# Autodesk Inventor assembly: Assembly
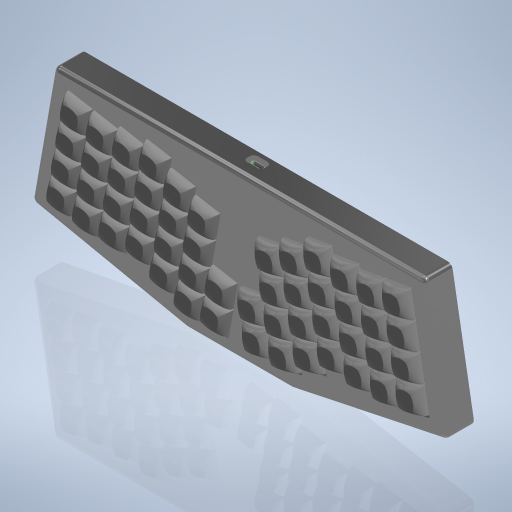
[picture p0: Inventor's stored thumbnail of the model, 512x512]
Saved by Autodesk Inventor 2023 (Build 270158000, 158)
## iProperties
Part Number: Assembly
Document SubType Name: Assembly
Designer: hainguyen
Author: hainguyen
## Documents named in this file (10)
- C:\Users\hainguyen\Documents\Inventor\atreus-52\Assembly.iam
- C:\Users\hainguyen\Documents\Inventor\atreus-52\atreus52_hotswap.ipt
- C:\Users\hainguyen\Documents\Inventor\atreus-52\Kailh Hotswap.ipt
- C:\Users\hainguyen\Documents\Inventor\atreus-52\asm_mx_asm_PLATE.ipt
- C:\Users\hainguyen\Documents\Inventor\atreus-52\DSA 1u.ipt
- C:\Users\hainguyen\Documents\Inventor\atreus-52\pattern.ipt
- C:\Users\hainguyen\Documents\Inventor\atreus-52\switch-plates.ipt
- C:\Users\hainguyen\Documents\Inventor\atreus-52\HRO_TYPE-C-31-M-12.ipt
- C:\Users\hainguyen\Documents\Inventor\atreus-52\bottom-case.ipt
- C:\Users\hainguyen\Documents\Inventor\atreus-52\top-case.ipt
## Components (162 placed, 9 different names)
1. atreus52_hotswap:1 — Mate:1, Mate:2, Mate:3, Mate:4, Mate:5, Angle:1, Mate:9, Mate:10, Mate:11, Mate:12, Mate:13, Angle:2, Flush:3, Mate:21, Mate:22
2. pattern:1 — Flush:1, Flush:2
3. switch-plates:1 — Mate:19, Mate:20, Flush:4
4. HRO_TYPE-C-31-M-12:1 — Flush:3, Mate:21, Mate:22
5. bottom-case:1 — Flush:4, Mate:23
6. top-case:1 — Mate:23
7. Kailh Hotswap:1 — Mate:1, Mate:2, Mate:3, Flush:1
8. asm_mx_asm_PLATE:1 — Mate:4, Mate:5, Angle:1, Mate:6, Mate:7, Mate:8
9. DSA 1u:1 — Mate:6, Mate:7, Mate:8
10. Kailh Hotswap:2
11. asm_mx_asm_PLATE:2
12. DSA 1u:2
13. Kailh Hotswap:3
14. asm_mx_asm_PLATE:3
15. DSA 1u:3
16. Kailh Hotswap:4
17. asm_mx_asm_PLATE:4
18. DSA 1u:4
19. Kailh Hotswap:5
20. asm_mx_asm_PLATE:5
21. DSA 1u:5
22. Kailh Hotswap:6
23. asm_mx_asm_PLATE:6
24. DSA 1u:6
25. Kailh Hotswap:7
26. asm_mx_asm_PLATE:7
27. DSA 1u:7
28. Kailh Hotswap:8
29. asm_mx_asm_PLATE:8
30. DSA 1u:8
31. Kailh Hotswap:9
32. asm_mx_asm_PLATE:9
33. DSA 1u:9
34. Kailh Hotswap:10
35. asm_mx_asm_PLATE:10
36. DSA 1u:10
37. Kailh Hotswap:11
38. asm_mx_asm_PLATE:11
39. DSA 1u:11
40. Kailh Hotswap:12
41. asm_mx_asm_PLATE:12
42. DSA 1u:12
43. Kailh Hotswap:13
44. asm_mx_asm_PLATE:13
45. DSA 1u:13
46. Kailh Hotswap:14
47. asm_mx_asm_PLATE:14
48. DSA 1u:14
49. Kailh Hotswap:15
50. asm_mx_asm_PLATE:15
51. DSA 1u:15
52. Kailh Hotswap:16
53. asm_mx_asm_PLATE:16
54. DSA 1u:16
55. Kailh Hotswap:17
56. asm_mx_asm_PLATE:17
57. DSA 1u:17
58. Kailh Hotswap:18
59. asm_mx_asm_PLATE:18
60. DSA 1u:18
61. Kailh Hotswap:19
62. asm_mx_asm_PLATE:19
63. DSA 1u:19
64. Kailh Hotswap:20
65. asm_mx_asm_PLATE:20
66. DSA 1u:20
67. Kailh Hotswap:21
68. asm_mx_asm_PLATE:21
69. DSA 1u:21
70. Kailh Hotswap:22
71. asm_mx_asm_PLATE:22
72. DSA 1u:22
73. Kailh Hotswap:23
74. asm_mx_asm_PLATE:23
75. DSA 1u:23
76. Kailh Hotswap:24
77. asm_mx_asm_PLATE:24
78. DSA 1u:24
79. Kailh Hotswap:25
80. asm_mx_asm_PLATE:25
81. DSA 1u:25
82. Kailh Hotswap:26
83. asm_mx_asm_PLATE:26
84. DSA 1u:26
85. asm_mx_asm_PLATE:27 — Mate:12, Mate:13, Angle:2, Mate:14, Mate:15, Mate:16, Mate:20
86. DSA 1u:27 — Mate:14, Mate:15, Mate:16
87. Kailh Hotswap:27 — Mate:9, Mate:10, Mate:11, Flush:2
88. asm_mx_asm_PLATE:28
89. DSA 1u:28
90. Kailh Hotswap:28
91. asm_mx_asm_PLATE:29
92. DSA 1u:29
93. Kailh Hotswap:29
94. asm_mx_asm_PLATE:30
95. DSA 1u:30
96. Kailh Hotswap:30
97. asm_mx_asm_PLATE:31
98. DSA 1u:31
99. Kailh Hotswap:31
100. asm_mx_asm_PLATE:32
101. DSA 1u:32
102. Kailh Hotswap:32
103. asm_mx_asm_PLATE:33
104. DSA 1u:33
105. Kailh Hotswap:33
106. asm_mx_asm_PLATE:34
107. DSA 1u:34
108. Kailh Hotswap:34
109. asm_mx_asm_PLATE:35
110. DSA 1u:35
111. Kailh Hotswap:35
112. asm_mx_asm_PLATE:36
113. DSA 1u:36
114. Kailh Hotswap:36
115. asm_mx_asm_PLATE:37
116. DSA 1u:37
117. Kailh Hotswap:37
118. asm_mx_asm_PLATE:38
119. DSA 1u:38
120. Kailh Hotswap:38
121. asm_mx_asm_PLATE:39
122. DSA 1u:39
123. Kailh Hotswap:39
124. asm_mx_asm_PLATE:40
125. DSA 1u:40
126. Kailh Hotswap:40
127. asm_mx_asm_PLATE:41
128. DSA 1u:41
129. Kailh Hotswap:41
130. asm_mx_asm_PLATE:42
131. DSA 1u:42
132. Kailh Hotswap:42
133. asm_mx_asm_PLATE:43
134. DSA 1u:43
135. Kailh Hotswap:43
136. asm_mx_asm_PLATE:44
137. DSA 1u:44
138. Kailh Hotswap:44
139. asm_mx_asm_PLATE:45
140. DSA 1u:45
141. Kailh Hotswap:45
142. asm_mx_asm_PLATE:46
143. DSA 1u:46
144. Kailh Hotswap:46
145. asm_mx_asm_PLATE:47
146. DSA 1u:47
147. Kailh Hotswap:47
148. asm_mx_asm_PLATE:48
149. DSA 1u:48
150. Kailh Hotswap:48
151. asm_mx_asm_PLATE:49
152. DSA 1u:49
153. Kailh Hotswap:49
154. asm_mx_asm_PLATE:50
155. DSA 1u:50
156. Kailh Hotswap:50
157. asm_mx_asm_PLATE:51
158. DSA 1u:51
159. Kailh Hotswap:51
160. asm_mx_asm_PLATE:52
161. DSA 1u:52
162. Kailh Hotswap:52
## Component patterns: (26 elements, first: Kailh Hotswap:1 + asm_mx_asm_PLATE:1 + DSA 1u:1), (26 elements, first: asm_mx_asm_PLATE:27 + DSA 1u:27 + Kailh Hotswap:27)
## Relationships (27: Mate 21, Flush 4, Angle 2)
- Mate:1: atreus52_hotswap:1 ↔ Kailh Hotswap:1
- Mate:2: atreus52_hotswap:1 ↔ Kailh Hotswap:1
- Mate:3: atreus52_hotswap:1 ↔ Kailh Hotswap:1
- Mate:4: atreus52_hotswap:1 ↔ asm_mx_asm_PLATE:1
- Mate:5: atreus52_hotswap:1 ↔ asm_mx_asm_PLATE:1
- Angle:1 (180 deg): atreus52_hotswap:1 ↔ asm_mx_asm_PLATE:1
- Mate:6: asm_mx_asm_PLATE:1 ↔ DSA 1u:1
- Mate:7: asm_mx_asm_PLATE:1 ↔ DSA 1u:1
- Mate:8: asm_mx_asm_PLATE:1 ↔ DSA 1u:1
- Flush:1: pattern:1 ↔ Kailh Hotswap:1
- Mate:9: atreus52_hotswap:1 ↔ Kailh Hotswap:27
- Mate:10: atreus52_hotswap:1 ↔ Kailh Hotswap:27
- Mate:11: atreus52_hotswap:1 ↔ Kailh Hotswap:27
- Mate:12: atreus52_hotswap:1 ↔ asm_mx_asm_PLATE:27
- Mate:13: atreus52_hotswap:1 ↔ asm_mx_asm_PLATE:27
- Angle:2 (180 deg): atreus52_hotswap:1 ↔ asm_mx_asm_PLATE:27
- Mate:14: asm_mx_asm_PLATE:27 ↔ DSA 1u:27
- Mate:15: asm_mx_asm_PLATE:27 ↔ DSA 1u:27
- Mate:16: asm_mx_asm_PLATE:27 ↔ DSA 1u:27
- Flush:2: pattern:1 ↔ Kailh Hotswap:27
- Flush:3: atreus52_hotswap:1 ↔ HRO_TYPE-C-31-M-12:1
- Mate:19: switch-plates:1
- Mate:20: switch-plates:1 ↔ asm_mx_asm_PLATE:27
- Flush:4: switch-plates:1 ↔ bottom-case:1
- Mate:21: atreus52_hotswap:1 ↔ HRO_TYPE-C-31-M-12:1
- Mate:22 (0.15 mm): atreus52_hotswap:1 ↔ HRO_TYPE-C-31-M-12:1
- Mate:23: bottom-case:1 ↔ top-case:1
